# Autodesk Inventor assembly: Assembly146-01
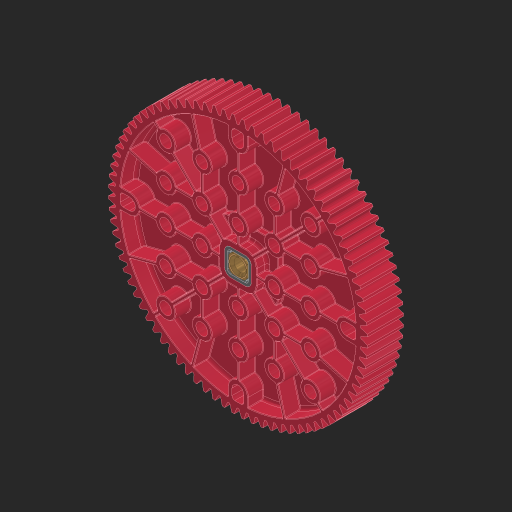
[picture p0: Inventor's stored thumbnail of the model, 512x512]
Saved by Autodesk Inventor 2023 (Build 270158000, 158)
## iProperties
Created: 2022-08-02
Part Number: Assembly146-01
Document SubType Name: Assembly
Designer: ylu12
Author: ylu12
## Documents named in this file (4)
- C:\Users\ylu12\Documents\GitHub\VEX-CAD-Inventor\Motion\Gears\HS Gear\HS 84T Gear, Circle.iam
- C:\Users\ylu12\Documents\GitHub\VEX-CAD-Inventor\Motion\HS Shaft Adapter Circle.ipt
- C:\Users\ylu12\Documents\GitHub\VEX-CAD-Inventor\Motion\Gears\Reference Files\HS 84T Gear, No Insert.ipt
- C:\Users\ylu12\Documents\GitHub\VEX-CAD-Inventor\Motion\Gears\HS Gear.iam
## Components (2 placed, 2 different names)
1. Circle — Mate:1, Mate:2, Flush:1
2. 84T — Flush:9, Mate:17, Mate:18
## Relationships (6: Mate 4, Flush 2)
- Mate:1: Circle
- Mate:2: Circle
- Flush:1 (6.35 mm): Circle
- Flush:9: 84T
- Mate:17: 84T
- Mate:18: 84T
